# Autodesk Inventor assembly: ScrapAssemblyRS3
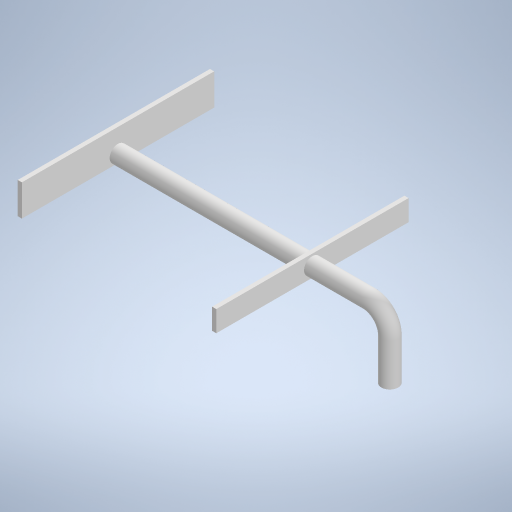
[picture p0: Inventor's stored thumbnail of the model, 512x512]
Saved by Autodesk Inventor 2024.3 (Build 283343000, 343)
## iProperties
Created: 2025-07-31
Part Number: ScrapAssemblyRS3
Document SubType Name: Assembly
Designer: ajclo
Author: ajclo
## Documents named in this file (4)
- C:\Users\ajclo\OneDrive - Stellenbosch University\Documents\BEng\Year IV\Skripsie\CAD\CAD Final Design\ScrapAssemblyRS3.iam
- C:\Users\ajclo\OneDrive - Stellenbosch University\Documents\BEng\Year IV\Skripsie\CAD\CAD Final Design\AllenKey-RS3.ipt
- C:\Users\ajclo\OneDrive - Stellenbosch University\Documents\BEng\Year IV\Skripsie\CAD\CAD Final Design\ScraperRS3.ipt
- C:\Users\ajclo\OneDrive - Stellenbosch University\Documents\BEng\Year IV\Skripsie\CAD\CAD Final Design\Scraper2RS3.ipt
## Components (3 placed, 3 different names)
1. AllenKey-RS3:1 — Mate:1, Tangent:1, Mate:2
2. ScraperRS3:1 — Mate:2, Flush:1, Flush:2
3. Scraper2RS3:1 — Mate:1, Tangent:1, Flush:1, Flush:2
## Relationships (5: Mate 2, Flush 2, Tangent 1)
- Mate:1: AllenKey-RS3:1 ↔ Scraper2RS3:1
- Tangent:1: AllenKey-RS3:1 ↔ Scraper2RS3:1
- Mate:2: AllenKey-RS3:1 ↔ ScraperRS3:1
- Flush:1: ScraperRS3:1 ↔ Scraper2RS3:1
- Flush:2 (93 mm): ScraperRS3:1 ↔ Scraper2RS3:1
